# Autodesk Inventor assembly: Assembly2
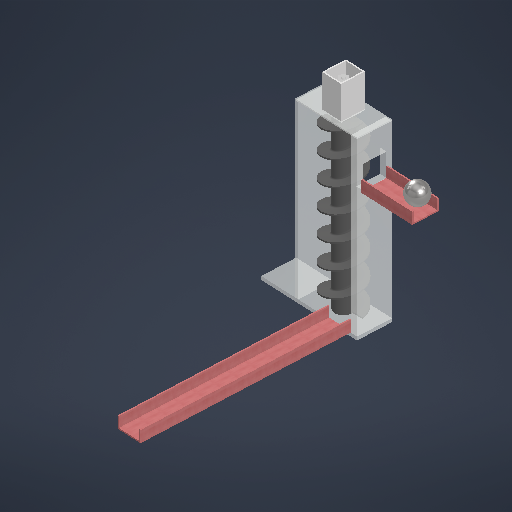
[picture p0: Inventor's stored thumbnail of the model, 512x512]
Saved by Autodesk Inventor 2026 (Build 300175000, 175)
## iProperties
Created: 2026-03-02
Part Number: Assembly2
Document SubType Name: Assembly
Designer: shahd
Author: shahd
## Documents named in this file (11)
- C:\Users\shahd\OneDrive - Faculty of Engineering Ain Shams University\BOM project\BOM project\Assembly2.iam
- C:\Users\shahd\OneDrive - Faculty of Engineering Ain Shams University\BOM project\BOM project\Part3.ipt
- C:\Users\shahd\OneDrive - Faculty of Engineering Ain Shams University\BOM project\BOM project\Part4.ipt
- C:\Users\shahd\OneDrive - Faculty of Engineering Ain Shams University\BOM project\BOM project\Lifting Mechanism.ipt
- C:\Users\shahd\OneDrive - Faculty of Engineering Ain Shams University\BOM project\BOM project\ball.ipt
- C:\Users\shahd\OneDrive - Faculty of Engineering Ain Shams University\BOM project\BOM project\base.ipt
- C:\Users\shahd\Downloads\slide1.ipt
- C:\Users\shahd\Downloads\slide2.ipt
- C:\Users\shahd\Downloads\partttt.ipt
- C:\Users\shahd\OneDrive - Faculty of Engineering Ain Shams University\BOM project\BOM project\motor box.ipt
- C:\Users\shahd\OneDrive - Faculty of Engineering Ain Shams University\BOM project\BOM project\Motor DC 16mm.ipt
## Components (13 placed, 10 different names)
1. Part3:1 — Mate:1, Mate:4, Flush:2, Mate:5, Mate:18, Flush:10
2. Part4:1 — Mate:1, Mate:4, Flush:2, Mate:7, Flush:3, Flush:4, Mate:9, Flush:5, Flush:6, Flush:7, Mate:21, Mate:22, Mate:23, Mate:24, Mate:25, Insert:1
3. Lifting Mechanism:1 — Mate:7, Mate:8, Mate:26
4. ball:1
5. base:1 — Mate:5, Mate:8, Flush:8, Mate:10, Mate:11, Mate:18, Flush:10
6. slide1:1 — Mate:10, Mate:11, Mate:12
7. slide2:1 — Mate:13, Mate:14, Mate:15, Mate:16, Flush:9, Mate:17
8. partttt:1 — Flush:3, Flush:4, Mate:9, Flush:5, Flush:6, Flush:7, Flush:8, Mate:12, Mate:13, Mate:14, Mate:15, Mate:16, Flush:9, Mate:17
9. motor box:1 — Mate:22, Mate:23, Flush:11, Flush:12
10. motor box:2 — Mate:21, Flush:13, Flush:14, Flush:15, Flush:16
11. motor box:4 — Mate:25, Flush:12, Flush:14, Flush:15
12. motor box:5 — Mate:24, Flush:11, Flush:13, Flush:16
13. Motor DC 16mm:1 — Mate:26, Insert:1
## Relationships (37: Mate 21, Flush 15, Insert 1)
- Mate:1: Part3:1 ↔ Part4:1
- Mate:4: Part3:1 ↔ Part4:1
- Flush:2: Part3:1 ↔ Part4:1
- Mate:5: Part3:1 ↔ base:1
- Mate:7: Part4:1 ↔ Lifting Mechanism:1
- Mate:8: Lifting Mechanism:1 ↔ base:1
- Flush:3: Part4:1 ↔ partttt:1
- Flush:4: Part4:1 ↔ partttt:1
- Mate:9: Part4:1 ↔ partttt:1
- Flush:5: Part4:1 ↔ partttt:1
- Flush:6: Part4:1 ↔ partttt:1
- Flush:7: Part4:1 ↔ partttt:1
- Flush:8: base:1 ↔ partttt:1
- Mate:10: base:1 ↔ slide1:1
- Mate:11: base:1 ↔ slide1:1
- Mate:12: slide1:1 ↔ partttt:1
- Mate:13: slide2:1 ↔ partttt:1
- Mate:14: slide2:1 ↔ partttt:1
- Mate:15: slide2:1 ↔ partttt:1
- Mate:16: slide2:1 ↔ partttt:1
- Flush:9: slide2:1 ↔ partttt:1
- Mate:17: slide2:1 ↔ partttt:1
- Mate:18: Part3:1 ↔ base:1
- Flush:10: Part3:1 ↔ base:1
- Mate:21: Part4:1 ↔ motor box:2
- Mate:22: Part4:1 ↔ motor box:1
- Mate:23: Part4:1 ↔ motor box:1
- Mate:24: Part4:1 ↔ motor box:5
- Mate:25: Part4:1 ↔ motor box:4
- Flush:11: motor box:1 ↔ motor box:5
- Flush:12: motor box:1 ↔ motor box:4
- Flush:13: motor box:2 ↔ motor box:5
- Flush:14: motor box:2 ↔ motor box:4
- Flush:15: motor box:2 ↔ motor box:4
- Flush:16: motor box:2 ↔ motor box:5
- Mate:26: Lifting Mechanism:1 ↔ Motor DC 16mm:1
- Insert:1: Part4:1 ↔ Motor DC 16mm:1
